# Autodesk Inventor assembly: Platinen-stack
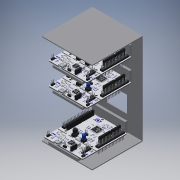
[picture p0: Inventor's stored thumbnail of the model, 180x180]
Saved by Autodesk Inventor 2017.3 (Build 213256000, 256)
## iProperties
Part Number: Platinen-stack
Material: Generisch
Document SubType Name: Assembly
Designer: Nils
Author: Nils
## Documents named in this file (4)
- C:\Users\Nils\Documents\GitHub\Eurobot2018\Hardware\Roboterplatform\Platinen-stack.iam
- C:\Users\Nils\Documents\GitHub\Eurobot2018\Hardware\Roboterplatform\Platinenhalter.ipt
- C:\Users\Nils\Documents\GitHub\Eurobot2018\Hardware\Roboterplatform\Platinenhalter-einzeln.ipt
- C:\Users\Nils\Documents\GitHub\Eurobot2018\Hardware\Roboterplatform\Nucleo-simplified\NUCLEO-F411RE-simplified.iam
## Components (7 placed, 3 different names)
1. Platinenhalter:1 — Fluchtend:1, Fluchtend:2, Fluchtend:3, Fluchtend:4, Fluchtend:5, Fluchtend:6, Passend:1, Passend:2, Fluchtend:7, Passend:3, Passend:4, Passend:5
2. Platinenhalter-einzeln:1 — Fluchtend:4, Fluchtend:7, Passend:3, Passend:6, Fluchtend:10
3. Platinenhalter-einzeln:2 — Fluchtend:5, Passend:2, Passend:5, Passend:7, Fluchtend:9
4. Platinenhalter-einzeln:3 — Fluchtend:6, Passend:1, Passend:4, Passend:8, Fluchtend:8
5. NUCLEO-F411RE-simplified:1 [sub-assembly] — Passend:7, Fluchtend:9, Fluchtend:13
6. NUCLEO-F411RE-simplified:2 [sub-assembly] — Passend:8, Fluchtend:8, Fluchtend:12
7. NUCLEO-F411RE-simplified:3 [sub-assembly] — Passend:6, Fluchtend:10, Fluchtend:11
## Relationships (21: Flush 13, Mate 8)
- Fluchtend:1 [Flush]: Platinenhalter:1
- Fluchtend:2 [Flush]: Platinenhalter:1
- Fluchtend:3 [Flush]: Platinenhalter:1
- Fluchtend:4 [Flush]: Platinenhalter:1 ↔ Platinenhalter-einzeln:1
- Fluchtend:5 [Flush]: Platinenhalter:1 ↔ Platinenhalter-einzeln:2
- Fluchtend:6 [Flush]: Platinenhalter:1 ↔ Platinenhalter-einzeln:3
- Passend:1 [Mate]: Platinenhalter:1 ↔ Platinenhalter-einzeln:3
- Passend:2 [Mate]: Platinenhalter:1 ↔ Platinenhalter-einzeln:2
- Fluchtend:7 [Flush] (-12 mm): Platinenhalter:1 ↔ Platinenhalter-einzeln:1
- Passend:3 [Mate] (7 mm): Platinenhalter:1 ↔ Platinenhalter-einzeln:1
- Passend:4 [Mate] (35 mm): Platinenhalter:1 ↔ Platinenhalter-einzeln:3
- Passend:5 [Mate] (75 mm): Platinenhalter:1 ↔ Platinenhalter-einzeln:2
- Passend:6 [Mate] (2 mm): Platinenhalter-einzeln:1 ↔ NUCLEO-F411RE-simplified:3
- Passend:7 [Mate] (2 mm): Platinenhalter-einzeln:2 ↔ NUCLEO-F411RE-simplified:1
- Passend:8 [Mate] (2 mm): Platinenhalter-einzeln:3 ↔ NUCLEO-F411RE-simplified:2
- Fluchtend:8 [Flush]: Platinenhalter-einzeln:3 ↔ NUCLEO-F411RE-simplified:2
- Fluchtend:9 [Flush]: Platinenhalter-einzeln:2 ↔ NUCLEO-F411RE-simplified:1
- Fluchtend:10 [Flush]: Platinenhalter-einzeln:1 ↔ NUCLEO-F411RE-simplified:3
- Fluchtend:11 [Flush]: NUCLEO-F411RE-simplified:3
- Fluchtend:12 [Flush]: NUCLEO-F411RE-simplified:2
- Fluchtend:13 [Flush]: NUCLEO-F411RE-simplified:1
